# Autodesk Inventor assembly: Pedestal Fixture Assembly
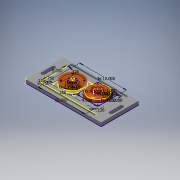
[picture p0: Inventor's stored thumbnail of the model, 180x180]
Saved by Autodesk Inventor 2018 (Build 220112000, 112)
## iProperties
Created: 2017-07-11
Part Number: Pedestal Fixture Assembly
Document SubType Name: Assembly
Designer: Samuel Clay
Author: Samuel Clay
## Documents named in this file (3)
- Z:\enclosure\inventor\Pedestal Fixture Assembly.iam
- Z:\enclosure\inventor\Pedestal Fixture Base.ipt
- Z:\enclosure\inventor\Pedestal.ipt
## Components (3 placed, 2 different names)
1. Pedestal Fixture Base:1 — Mate:1, Mate:2, Mate:3, Mate:7, Mate:8, Mate:9, Mate:10
2. Pedestal:1 — Mate:7, Mate:8, Mate:9, Mate:10
3. Pedestal:2 — Mate:1, Mate:2, Mate:3
## Relationships (7: Mate 7)
- Mate:1 (0.635 mm): Pedestal Fixture Base:1 ↔ Pedestal:2
- Mate:2 (2.54 mm): Pedestal Fixture Base:1 ↔ Pedestal:2
- Mate:3 (1.27 mm): Pedestal Fixture Base:1 ↔ Pedestal:2
- Mate:7 (19.05 mm): Pedestal Fixture Base:1 ↔ Pedestal:1
- Mate:8 (6.35 mm): Pedestal Fixture Base:1 ↔ Pedestal:1
- Mate:9 (15.24 mm): Pedestal Fixture Base:1 ↔ Pedestal:1
- Mate:10 (-6.35 mm): Pedestal Fixture Base:1 ↔ Pedestal:1
